# Autodesk Inventor assembly: E3Dv6 Alone
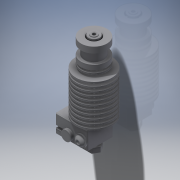
[picture p0: Inventor's stored thumbnail of the model, 180x180]
Saved by Autodesk Inventor 2016 SP1 (Build 200210100, 210)
## iProperties
Created: 2015-05-11
Part Number: E3Dv6 Alone
Document SubType Name: Assembly
Designer: Mathias Lyngklip Kjeldgaard
Mass: 11.6284 g
Surface Area: 152.251 cm^2
Volume: 11.6284 cm^3
Density: 1 g/cm^3
Author: Mike
Title: E3D v6.STEP
Description: STEP AP203
Creation Date: 2015-02-14
Sending System: SolidWorks 2013
Preprocessor: SwSTEP 2.0
Author: Mathias Lyngklip Kjeldgaard
## Documents named in this file (12)
- C:\Users\PowerStation9000\AppData\Local\Autodesk\Autodesk Sync\Cloud\mathiaslk\UltiBot mk2\Importerede komponenter\E3Dv6 Hotend\E3Dv6 Alone.iam
- C:\Users\PowerStation9000\AppData\Local\Autodesk\Autodesk Sync\Cloud\mathiaslk\UltiBot mk2\Importerede komponenter\E3Dv6 Hotend\v6 Heatsink.ipt
- C:\Users\PowerStation9000\AppData\Local\Autodesk\Autodesk Sync\Cloud\mathiaslk\UltiBot mk2\Importerede komponenter\E3Dv6 Hotend\v6 Heatbreak.ipt
- C:\Users\PowerStation9000\AppData\Local\Autodesk\Autodesk Sync\Cloud\mathiaslk\UltiBot mk2\Importerede komponenter\E3Dv6 Hotend\v6 Heat Block.ipt
- C:\Users\PowerStation9000\AppData\Local\Autodesk\Autodesk Sync\Cloud\mathiaslk\UltiBot mk2\Importerede komponenter\E3Dv6 Hotend\v6 Nozzle_.4.ipt
- C:\Users\PowerStation9000\AppData\Local\Autodesk\Autodesk Sync\Cloud\mathiaslk\UltiBot mk2\Importerede komponenter\E3Dv6 Hotend\v6 Ferrule.ipt
- C:\Users\PowerStation9000\AppData\Local\Autodesk\Autodesk Sync\Cloud\mathiaslk\UltiBot mk2\Importerede komponenter\E3Dv6 Hotend\v6 Coupling.ipt
- C:\Users\PowerStation9000\AppData\Local\Autodesk\Autodesk Sync\Cloud\mathiaslk\UltiBot mk2\Importerede komponenter\E3Dv6 Hotend\PTFE Tube.ipt
- C:\Users\PowerStation9000\AppData\Local\Autodesk\Autodesk Sync\Cloud\mathiaslk\UltiBot mk2\Importerede komponenter\E3Dv6 Hotend\cartridge heater.ipt
- C:\Users\PowerStation9000\AppData\Local\Autodesk\Autodesk Sync\Cloud\mathiaslk\UltiBot mk2\Importerede komponenter\E3Dv6 Hotend\socket button head cap screw_am_B18.3.4M - 3 x 0.5 x 3 SBHCS --N.ipt
- C:\Users\PowerStation9000\AppData\Local\Autodesk\Autodesk Sync\Cloud\mathiaslk\UltiBot mk2\Importerede komponenter\E3Dv6 Hotend\socket button head cap screw_am_B18.3.4M - 3 x 0.5 x 12 SBHCS --S.ipt
- C:\Users\PowerStation9000\AppData\Local\Autodesk\Autodesk Sync\Cloud\mathiaslk\UltiBot mk2\Importerede komponenter\E3Dv6 Hotend\flat washer narrow_am_B18.22M - Plain washer, 3 mm, narrow.ipt
## Components (11 placed, 11 different names)
1. v6 Heatsink_1 — Mate:13, Flush:2, Mate:21, Mate:22, Mate:25
2. v6 Heatbreak_2 — Mate:13, Flush:2, Mate:14, Mate:15, Mate:16, Flush:3, Mate:23
3. v6 Heat Block_3 — Mate:14, Flush:3, Mate:17, Mate:18, Flush:4, Mate:19, Mate:26, Mate:27, Mate:28, Angle:2, Angle:3
4. v6 Nozzle_.4_4 — Mate:15, Mate:16, Angle:2
5. v6 Ferrule_5 — Mate:20, Mate:21, Mate:22
6. v6 Coupling_6 — Mate:24, Mate:25
7. PTFE Tube_7 — Mate:20, Mate:23, Mate:24
8. cartridge heater_14 — Mate:17, Flush:4
9. socket button head cap screw_am_B18.3.4M - 3 x 0.5 x 3 SBHCS --N_15 — Mate:27, Mate:29
10. socket button head cap screw_am_B18.3.4M - 3 x 0.5 x 12 SBHCS --S_16 — Mate:18, Mate:19
11. flat washer narrow_am_B18.22M - Plain washer, 3 mm, narrow_17 — Mate:26, Mate:28, Mate:29
## Relationships (22: Mate 17, Flush 3, Angle 2)
- Mate:13: v6 Heatsink_1 ↔ v6 Heatbreak_2
- Flush:2: v6 Heatsink_1 ↔ v6 Heatbreak_2
- Mate:14: v6 Heatbreak_2 ↔ v6 Heat Block_3
- Mate:15: v6 Heatbreak_2 ↔ v6 Nozzle_.4_4
- Mate:16: v6 Heatbreak_2 ↔ v6 Nozzle_.4_4
- Flush:3: v6 Heatbreak_2 ↔ v6 Heat Block_3
- Mate:17: v6 Heat Block_3 ↔ cartridge heater_14
- Mate:18: v6 Heat Block_3 ↔ socket button head cap screw_am_B18.3.4M - 3 x 0.5 x 12 SBHCS --S_16
- Flush:4 (1.867 mm): v6 Heat Block_3 ↔ cartridge heater_14
- Mate:19: v6 Heat Block_3 ↔ socket button head cap screw_am_B18.3.4M - 3 x 0.5 x 12 SBHCS --S_16
- Mate:20: v6 Ferrule_5 ↔ PTFE Tube_7
- Mate:21: v6 Heatsink_1 ↔ v6 Ferrule_5
- Mate:22: v6 Heatsink_1 ↔ v6 Ferrule_5
- Mate:23: v6 Heatbreak_2 ↔ PTFE Tube_7
- Mate:24: v6 Coupling_6 ↔ PTFE Tube_7
- Mate:25: v6 Heatsink_1 ↔ v6 Coupling_6
- Mate:26: v6 Heat Block_3 ↔ flat washer narrow_am_B18.22M - Plain washer, 3 mm, narrow_17
- Mate:27: v6 Heat Block_3 ↔ socket button head cap screw_am_B18.3.4M - 3 x 0.5 x 3 SBHCS --N_15
- Mate:28: v6 Heat Block_3 ↔ flat washer narrow_am_B18.22M - Plain washer, 3 mm, narrow_17
- Mate:29: socket button head cap screw_am_B18.3.4M - 3 x 0.5 x 3 SBHCS --N_15 ↔ flat washer narrow_am_B18.22M - Plain washer, 3 mm, narrow_17
- Angle:2 (0 deg): v6 Heat Block_3 ↔ v6 Nozzle_.4_4
- Angle:3 (0 deg): v6 Heat Block_3
